# Autodesk Inventor assembly: YagiFront
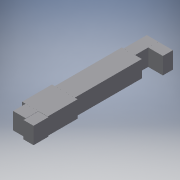
[picture p0: Inventor's stored thumbnail of the model, 180x180]
Saved by Autodesk Inventor 2016 (Build 200138000, 138)
## iProperties
Created: 2016-08-31
Part Number: YagiFront
Document SubType Name: Assembly
Designer: jfixelle
Author: jfixelle
## Documents named in this file (6)
- E:\jfixelle\Documents\APC\GitRepo\FrontEnd\Placement\YagiFront.iam
- E:\jfixelle\Documents\APC\GitRepo\FrontEnd\Placement\AmplifierBlock1.ipt
- E:\jfixelle\Documents\APC\GitRepo\FrontEnd\Placement\AmplifierBlock2.ipt
- E:\jfixelle\Documents\APC\GitRepo\FrontEnd\Placement\CouplerBlock.ipt
- E:\jfixelle\Documents\APC\GitRepo\FrontEnd\Placement\FilterBlock.ipt
- E:\jfixelle\Documents\APC\GitRepo\FrontEnd\Placement\UMCCBlock.ipt
## Components (6 placed, 5 different names)
1. AmplifierBlock1:1 — Flush:1, Flush:2, Flush:3, Flush:4, Flush:6
2. AmplifierBlock2:1 — Flush:2
3. CouplerBlock:1 — Flush:4
4. FilterBlock:1 — Flush:1
5. UMCCBlock:1 — Flush:6
6. UMCCBlock:2 — Flush:3
## Relationships (5: Flush 5)
- Flush:1: AmplifierBlock1:1 ↔ FilterBlock:1
- Flush:2: AmplifierBlock1:1 ↔ AmplifierBlock2:1
- Flush:3: AmplifierBlock1:1 ↔ UMCCBlock:2
- Flush:4: AmplifierBlock1:1 ↔ CouplerBlock:1
- Flush:6: AmplifierBlock1:1 ↔ UMCCBlock:1
